# Autodesk Inventor assembly: dec_bot_design
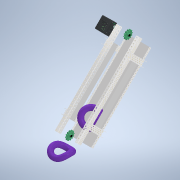
[picture p0: Inventor's stored thumbnail of the model, 180x180]
Saved by Autodesk Inventor 2022 (Build 260153000, 153)
## iProperties
Created: 2021-11-22
Part Number: dec_bot_design
Document SubType Name: Assembly
Designer: Alex
Author: Alex
## Documents named in this file (9)
- C:\Users\Alex\Documents\robotics\cad\DecBot\333B\dec_bot_design.iam
- C:\Users\Alex\Documents\robotics\cad\Library 1.2\Structure\C-Channels\Aluminum 1x2x1\1x2x1x35 Aluminum.ipt
- C:\Users\Alex\Documents\robotics\cad\Library 1.2\Electronics\V5 Motor.ipt
- C:\Users\Alex\Documents\robotics\cad\Tipping Poing Field CAD\Ring.ipt
- C:\Users\Alex\Documents\robotics\cad\Library 1.2\Motion\Sprockets\HS 12T Sprocket, Square.ipt
- C:\Users\Alex\Documents\robotics\cad\Library 1.2\Structure\C-Channels\Aluminum 1x2x1\1x2x1x8 Aluminum.ipt
- C:\Users\Alex\Documents\robotics\cad\Library 1.2\Structure\C-Channels\Aluminum 1x2x1 Half\1x2x1x33 Aluminum Half.ipt
- C:\Users\Alex\Documents\robotics\cad\DecBot\333B\lexan_pieces\conveyorv2_backing.ipt
- C:\Users\Alex\Documents\robotics\cad\DecBot\333B\lexan_pieces\conveyorv2_siding.ipt
## Components (16 placed, 8 different names)
1. Ring:2
2. V5 Motor:2
3. 1x2x1x35 Aluminum:8 — Insert:57, Insert:58
4. 1x2x1x8 Aluminum:5 — Insert:55, Insert:56
5. 1x2x1x8 Aluminum:6 — Insert:41, Insert:42
6. 1x2x1x33 Aluminum Half:1 — Insert:41, Insert:42, Insert:49, Insert:50
7. 1x2x1x35 Aluminum:9
8. 1x2x1x8 Aluminum:7 — Insert:47, Insert:48, Insert:53, Insert:54
9. 1x2x1x8 Aluminum:8
10. 1x2x1x33 Aluminum Half:2 — Insert:47, Insert:48, Insert:51, Insert:52
11. conveyorv2_backing:1 — Insert:49, Insert:50, Insert:51, Insert:52
12. Ring:3
13. conveyorv2_siding:1 — Insert:53, Insert:54
14. conveyorv2_siding:2 — Insert:55, Insert:56
15. HS 12T Sprocket, Square:3 — Insert:57
16. HS 12T Sprocket, Square:4 — Insert:58
## Relationships (24: Insert 24)
- [Insert]: V5 Motor:2 ↔ 1x2x1x35 Aluminum:8
- [Insert]: V5 Motor:2 ↔ 1x2x1x35 Aluminum:8
- [Insert]: 1x2x1x35 Aluminum:8 ↔ 1x2x1x8 Aluminum:5
- [Insert]: 1x2x1x35 Aluminum:8 ↔ 1x2x1x8 Aluminum:5
- [Insert]: 1x2x1x35 Aluminum:8 ↔ 1x2x1x8 Aluminum:6
- [Insert]: 1x2x1x35 Aluminum:8 ↔ 1x2x1x8 Aluminum:6
- Insert:41: 1x2x1x8 Aluminum:6 ↔ 1x2x1x33 Aluminum Half:1
- Insert:42: 1x2x1x8 Aluminum:6 ↔ 1x2x1x33 Aluminum Half:1
- [Insert]: 1x2x1x35 Aluminum:9 ↔ 1x2x1x8 Aluminum:7
- [Insert]: 1x2x1x35 Aluminum:9 ↔ 1x2x1x8 Aluminum:7
- [Insert]: 1x2x1x35 Aluminum:9 ↔ 1x2x1x8 Aluminum:8
- [Insert]: 1x2x1x35 Aluminum:9 ↔ 1x2x1x8 Aluminum:8
- Insert:47: 1x2x1x8 Aluminum:7 ↔ 1x2x1x33 Aluminum Half:2
- Insert:48: 1x2x1x8 Aluminum:7 ↔ 1x2x1x33 Aluminum Half:2
- Insert:49: 1x2x1x33 Aluminum Half:1 ↔ conveyorv2_backing:1
- Insert:50: 1x2x1x33 Aluminum Half:1 ↔ conveyorv2_backing:1
- Insert:51: 1x2x1x33 Aluminum Half:2 ↔ conveyorv2_backing:1
- Insert:52: 1x2x1x33 Aluminum Half:2 ↔ conveyorv2_backing:1
- Insert:53: 1x2x1x8 Aluminum:7 ↔ conveyorv2_siding:1
- Insert:54: 1x2x1x8 Aluminum:7 ↔ conveyorv2_siding:1
- Insert:55: 1x2x1x8 Aluminum:5 ↔ conveyorv2_siding:2
- Insert:56: 1x2x1x8 Aluminum:5 ↔ conveyorv2_siding:2
- Insert:57 (50.8 mm): 1x2x1x35 Aluminum:8 ↔ HS 12T Sprocket, Square:3
- Insert:58 (50.8 mm): 1x2x1x35 Aluminum:8 ↔ HS 12T Sprocket, Square:4
## Named parameters: d48_d30 = 0 mm, d49_d31 = 0 mm, d50_d32 = 0 mm, d51_d33 = 0 mm, d52_d16 = 0 mm, d53_d17 = 0 mm, d56_d22 = 0 mm, d57_d23 = 0 mm, d58_d26 = 0 mm, d59_d27 = 0 mm
